# Autodesk Inventor assembly: 1103 Lift - BottomTier
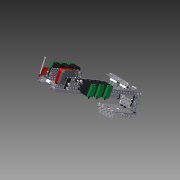
[picture p0: Inventor's stored thumbnail of the model, 180x180]
Saved by Autodesk Inventor 2012 (Build 160160000, 160)
## iProperties
Created: 2011-08-16
Part Number: 1103 Lift - BottomTier
Document SubType Name: Assembly
Designer: Dakota.Bayer
Author: Dakota.Bayer
## Documents named in this file (37)
- C:\Users\Wade\Documents\1103 Robot - CAD Assembly\1103 Lift - Bottom Tier.iam
- C:\Users\Wade\Documents\1103 Robot - CAD Assembly\Outside.ipt
- C:\Users\Wade\Documents\1103 Robot - CAD Assembly\Flat Bearing Block.ipt
- C:\Users\Wade\Documents\1103 Robot - CAD Assembly\2 x 12.ipt
- C:\Users\Wade\Documents\1103 Robot - CAD Assembly\1103 lift base.ipt
- C:\Users\Wade\Documents\24C VEX CAD Files\Washers & Spacers\Spacer (Nylon), 0.125''.ipt
- C:\Users\Wade\Documents\24C VEX CAD Files\Motors & Sensors\Optical Shaft (Quadrature) Encoder.iam
- C:\Users\Wade\Documents\24C VEX CAD Files\Standoffs & Couplers\Standoff 2.40''.ipt
- C:\Users\Wade\Documents\24C VEX CAD Files\Screws & Nuts\Screw 6-32 x 0.250''-Silver.ipt
- C:\Users\Wade\Documents\1103 Robot - CAD Assembly\Bearing Assembly (end hole).iam
- C:\Users\Wade\Documents\1103 Robot - CAD Assembly\Bearing Assembly (both end holes).iam
- C:\Users\Wade\Documents\24C VEX CAD Files\Screws & Nuts\Screw 8-32 x 0.875''-Silver.ipt
- C:\Users\Wade\Documents\24C VEX CAD Files\Screws & Nuts\Nut 8-32 Nylock.ipt
- C:\Users\Wade\Documents\24C VEX CAD Files\Screws & Nuts\Screw 8-32 x 0.500''-Silver.ipt
- C:\Users\Wade\Documents\1103 Robot - CAD Assembly\BEAM-0500.ipt
- C:\Users\Wade\Documents\24C VEX CAD Files\Motors & Sensors\2-Wire Motor 269-Without Wire.iam
- C:\Users\Wade\Documents\1103 Robot - CAD Assembly\VEX-HINGE-2 RevA_1.ipt
- C:\Users\Wade\Documents\1103 Robot - CAD Assembly\1103 sprocket4.ipt
- C:\Users\Wade\Documents\1103 Robot - CAD Assembly\1103 sprocket3.ipt
- C:\Users\Wade\Documents\1103 Robot - CAD Assembly\5 x 2.ipt
- C:\Users\Wade\Documents\1103 Robot - CAD Assembly\1103 sprocket1.ipt
- C:\Users\Wade\Documents\1103 Robot - CAD Assembly\1103 sprocket2.ipt
- C:\Users\Wade\Documents\24C VEX CAD Files\Screws & Nuts\Screw 8-32 x 0.375''-Silver.ipt
- C:\Users\Wade\Documents\1103 Robot - CAD Assembly\.375'' Screw & Nylock Nut.iam
- C:\Users\Wade\Documents\24C VEX CAD Files\Screws & Nuts\Screw 8-32 x 0.250''-Silver.ipt
- C:\Users\Wade\Documents\24C VEX CAD Files\Screws & Nuts\Nut 8-32 Keps.ipt
- C:\Users\Wade\Documents\24C VEX CAD Files\Metal Chassis Rails\Aluminum Chassis Rail 2x1x5.ipt
- C:\Users\Wade\Documents\24C VEX CAD Files\Motors & Sensors\Limit Switch (Sensor).iam
- C:\Users\Wade\Documents\24C VEX CAD Files\Washers & Spacers\Spacer (Thin), 4.6mm.ipt
- C:\Users\Wade\Documents\24C VEX CAD Files\Washers & Spacers\Spacer (Nylon), 0.250''.ipt
- C:\Users\Wade\Documents\24C VEX CAD Files\Standoffs & Couplers\Standoff 0.75''.ipt
- C:\Users\Wade\Documents\24C VEX CAD Files\Screws & Nuts\Screw 6-32 x 0.500''-Silver.ipt
- C:\Users\Wade\Documents\1103 Robot - CAD Assembly\VEX-HINGE 4x RevA.ipt
- C:\Users\Wade\Documents\24C VEX CAD Files\Washers & Spacers\Spacer (Nylon), 0.500'' (mod).ipt
- C:\Users\Wade\Documents\24C VEX CAD Files\Washers & Spacers\Spacer (Nylon), 0.250'' (mod).ipt
- C:\Users\Wade\Documents\24C VEX CAD Files\Other Parts\Bearing Flat (2-hole).ipt
- C:\Users\Wade\Documents\1103 Robot - CAD Assembly\.5'' Screw & Nylock Nut.iam
## Components (141 placed, 36 different names)
1. Outside:3 — Flush:21, Flush:23, Mate:622, Mate:685
2. Outside:4 — Mate:54, Flush:23, Flush:35, Mate:686
3. 1103 lift base:1 — Mate:54, Flush:21, Mate:112, Mate:113, Flush:29, Flush:30, Flush:31, Flush:32, Mate:622, Flush:35, Tangent:152, Mate:633, Tangent:153, Flush:36, Mate:638, Mate:640, Mate:655, Mate:660, Mate:689, Mate:690, Mate:693, Flush:38, Mate:694, Flush:39, Flush:40, Tangent:177, Mate:784, Tangent:219, Tangent:220, Mate:790, Mate:791, Mate:792, Mate:793, Mate:798, Mate:799, Mate:800, Mate:801, Tangent:222, Tangent:223, Tangent:224, Mate:804, Mate:806, Mate:810, Mate:820, Angle:1, Angle:2, Mate:835, Mate:839
4. Screw 8-32 x 0.375''-Silver:1 — Mate:683
5. Screw 8-32 x 0.375''-Silver:2 — Mate:684
6. Screw 8-32 x 0.375''-Silver:3 — Mate:688
7. Screw 8-32 x 0.375''-Silver:4 — Mate:687
8. 2 x 12:1 — Mate:112, Flush:29, Flush:32, Mate:114, Tangent:154, Tangent:155, Tangent:156, Mate:641, Tangent:157, Tangent:158, Tangent:159, Tangent:160, Tangent:161, Mate:644, Mate:661, Mate:674, Mate:675, Mate:676, Mate:816, Mate:817
9. 2 x 12:2 — Mate:113, Flush:30, Flush:31, Mate:119, Mate:625, Mate:645, Mate:648, Tangent:162, Tangent:163, Tangent:164, Tangent:165, Tangent:166, Mate:649, Tangent:167, Mate:654, Mate:667, Mate:668, Mate:669, Mate:818
10. Flat Bearing Block:5 — Mate:114, Mate:664, Flush:37, Mate:741
11. Screw 8-32 x 0.500''-Silver:1 — Mate:661, Mate:662
12. Screw 8-32 x 0.500''-Silver:2 — Mate:660, Mate:663
13. Screw 8-32 x 0.500''-Silver:3 — Mate:654, Mate:657
14. Screw 8-32 x 0.500''-Silver:4 — Mate:655, Mate:656
15. Flat Bearing Block:6 — Mate:119, Mate:658, Mate:659
16. Screw 8-32 x 0.875''-Silver:1 — Mate:691
17. Screw 6-32 x 0.500''-Silver:1
18. Screw 6-32 x 0.500''-Silver:2
19. Screw 6-32 x 0.500''-Silver:3
20. Screw 6-32 x 0.500''-Silver:4
21. Bearing Assembly (end hole):2 [sub-assembly] — Tangent:157, Tangent:158, Mate:816, Mate:817
22. Screw 6-32 x 0.500''-Silver:5
23. Screw 6-32 x 0.500''-Silver:6
24. Screw 6-32 x 0.500''-Silver:7
25. Screw 6-32 x 0.500''-Silver:8
26. Screw 6-32 x 0.500''-Silver:9
27. Screw 6-32 x 0.500''-Silver:10
28. Screw 6-32 x 0.500''-Silver:11
29. Screw 6-32 x 0.500''-Silver:12
30. Spacer (Nylon), 0.125'':1 — Mate:625, Mate:632
31. Optical Shaft (Quadrature) Encoder:1 [sub-assembly] — Mate:632
32. Standoff 2.40'':1 — Tangent:152, Mate:633, Tangent:153, Mate:637, Mate:639
33. Spacer (Nylon), 0.500'' (mod):1 — Flush:36
34. Screw 6-32 x 0.250''-Silver:1 — Mate:639, Mate:640
35. Screw 6-32 x 0.250''-Silver:2 — Mate:637, Mate:638
36. Bearing Assembly (end hole):1 [sub-assembly] — Tangent:154, Tangent:155, Tangent:156, Mate:641
37. Bearing Assembly (end hole):3 [sub-assembly] — Tangent:159, Tangent:160, Tangent:161, Mate:644, Mate:647
38. Bearing Assembly (end hole):5 [sub-assembly] — Mate:648, Tangent:162, Tangent:163, Tangent:164
39. Bearing Assembly (end hole):6 [sub-assembly] — Tangent:165, Tangent:166, Mate:649, Tangent:167
40. Bearing Assembly (both end holes):1 [sub-assembly] — Mate:645, Mate:647, Mate:692, Mate:818
41. Nut 8-32 Nylock:3 — Mate:657, Mate:658
42. Nut 8-32 Nylock:4 — Mate:656, Mate:659
43. BEAM-0500:1 — Mate:662, Flush:37, Mate:740, Mate:742
44. BEAM-0500:2 — Mate:663, Mate:664, Mate:743
45. 2-Wire Motor 269-Without Wire:1 [sub-assembly] — Mate:667
46. 2-Wire Motor 269-Without Wire:2 [sub-assembly] — Mate:669
47. 2-Wire Motor 269-Without Wire:3 [sub-assembly] — Mate:668
48. 2-Wire Motor 269-Without Wire:4 [sub-assembly] — Mate:675
49. 2-Wire Motor 269-Without Wire:5 [sub-assembly] — Mate:676
50. 2-Wire Motor 269-Without Wire:6 [sub-assembly] — Mate:674
51. VEX-HINGE 4x RevA:1 — Mate:802, Mate:803, Mate:822, Angle:2
52. VEX-HINGE-2 RevA_1:1 — Mate:747, Flush:54, Flush:55, Mate:750, Tangent:207, Tangent:209, Tangent:210, Mate:751, Mate:802, Mate:803
53. 1103 sprocket4:1 — Mate:694, Flush:39, Tangent:171, Tangent:172, Tangent:173, Mate:697, Mate:701, Mate:703, Flush:41, Mate:704, Flush:42, Tangent:178, Mate:705, Tangent:179, Tangent:180, Tangent:181
54. 1103 sprocket3:1 — Mate:693, Flush:38, Flush:40, Tangent:168, Tangent:169, Mate:696, Tangent:170, Tangent:174, Tangent:175, Mate:698, Tangent:176, Mate:699, Mate:707, Tangent:182, Tangent:183, Mate:819
55. 5 x 2:1 — Mate:747, Flush:54, Flush:55, Tangent:205, Tangent:206, Tangent:208, Tangent:211, Tangent:212, Tangent:213, Tangent:214, Tangent:215, Tangent:216, Tangent:217, Tangent:218, Mate:776, Mate:777, Mate:778, Mate:779, Mate:780, Mate:782, Mate:783, Mate:785, Mate:821, Mate:822, Angle:1
56. 1103 sprocket1:1 — Mate:709, Flush:43, Flush:44, Mate:722, Tangent:194, Tangent:195, Mate:723, Mate:727, Tangent:198, Tangent:199, Mate:730, Tangent:201, Mate:731, Mate:738, Mate:739
57. 1103 sprocket2:1 — Mate:710, Flush:45, Flush:46, Flush:48, Flush:49, Mate:728, Mate:729, Tangent:196, Tangent:197, Tangent:200, Tangent:202, Mate:736, Mate:737, Mate:831
58. 5 x 2:2 — Flush:41, Mate:704, Flush:42, Tangent:184, Tangent:185, Mate:709, Flush:43, Flush:44, Mate:710, Flush:45, Flush:46, Mate:706, Mate:708, Mate:715, Mate:717, Mate:719, Mate:721, Mate:819, Mate:827, Mate:828, Mate:829, Mate:830
59. Nut 8-32 Nylock:5 — Mate:684, Mate:686
60. Nut 8-32 Nylock:6 — Mate:683, Mate:685
61. Nut 8-32 Nylock:7 — Mate:688, Mate:689
62. Nut 8-32 Nylock:8 — Mate:687, Mate:690
63. Nut 8-32 Nylock:9 — Mate:691, Mate:692
64. Bearing Assembly (both end holes):2 [sub-assembly] — Tangent:168, Tangent:169, Mate:696, Tangent:170
65. Bearing Assembly (both end holes):3 [sub-assembly] — Tangent:171, Tangent:172, Tangent:173, Mate:697
66. .375'' Screw & Nylock Nut:1 [sub-assembly] — Tangent:176, Tangent:177, Mate:699, Mate:700
67. .375'' Screw & Nylock Nut:2 [sub-assembly] — Mate:702, Mate:703
68. .375'' Screw & Nylock Nut:3 [sub-assembly] — Mate:700, Mate:701
69. .375'' Screw & Nylock Nut:4 [sub-assembly] — Tangent:174, Tangent:175, Mate:698, Mate:702
70. .375'' Screw & Nylock Nut:5 [sub-assembly] — Tangent:178, Mate:705, Tangent:179
71. .375'' Screw & Nylock Nut:6 [sub-assembly] — Mate:706, Tangent:180, Tangent:181
72. .375'' Screw & Nylock Nut:7 [sub-assembly] — Mate:707, Tangent:184, Tangent:185
73. .375'' Screw & Nylock Nut:8 [sub-assembly] — Mate:708, Tangent:182, Tangent:183
74. Screw 8-32 x 0.375''-Silver:5
75. Screw 8-32 x 0.375''-Silver:6 — Mate:831
76. Screw 8-32 x 0.375''-Silver:8
77. Screw 8-32 x 0.375''-Silver:7
78. Nut 8-32 Keps:1 — Mate:715
79. Nut 8-32 Keps:2 — Mate:721
80. Nut 8-32 Keps:3 — Mate:719
81. Nut 8-32 Keps:4 — Mate:717
82. Aluminum Chassis Rail 2x1x5:1 — Flush:48, Mate:722, Flush:49, Flush:50
83. .375'' Screw & Nylock Nut:9 [sub-assembly] — Tangent:194, Tangent:195, Mate:723
84. .375'' Screw & Nylock Nut:10 [sub-assembly] — Mate:725, Mate:727, Tangent:198
85. .375'' Screw & Nylock Nut:11 [sub-assembly] — Mate:724, Mate:729, Tangent:196
86. .375'' Screw & Nylock Nut:12 [sub-assembly] — Mate:726, Mate:728, Tangent:197
87. Standoff 2.40'':2 — Tangent:199, Mate:730, Tangent:200, Mate:732, Mate:735
88. Standoff 2.40'':3 — Tangent:201, Tangent:202, Mate:731, Mate:733, Mate:734
89. Screw 8-32 x 0.250''-Silver:5 — Mate:733, Mate:738
90. Screw 8-32 x 0.250''-Silver:6 — Mate:732, Mate:739
91. Screw 8-32 x 0.250''-Silver:7 — Mate:734, Mate:736
92. Screw 8-32 x 0.250''-Silver:8 — Mate:735, Mate:737
93. Limit Switch (Sensor):1 [sub-assembly] — Mate:740, Mate:741, Mate:744, Mate:745
94. Screw 8-32 x 0.500''-Silver:5 — Mate:743, Mate:745
95. Screw 8-32 x 0.500''-Silver:6 — Mate:742, Mate:744
96. Spacer (Thin), 4.6mm:1 — Flush:59, Mate:752, Mate:766, Mate:771
97. Spacer (Nylon), 0.250'':1 — Tangent:211, Tangent:212, Flush:59, Mate:754, Mate:764, Mate:821
98. Spacer (Thin), 4.6mm:2 — Tangent:205, Tangent:206, Flush:58, Mate:753, Mate:772, Mate:781
99. Spacer (Nylon), 0.250'' (mod):1 — Tangent:213, Tangent:214, Flush:58, Mate:755, Mate:765
100. Spacer (Thin), 4.6mm:3 — Tangent:207, Tangent:208, Mate:750, Flush:57, Mate:756, Mate:763, Mate:773
101. Spacer (Nylon), 0.250'':3 — Tangent:217, Tangent:218, Flush:56, Mate:759, Mate:760, Mate:767
102. Spacer (Thin), 4.6mm:4 — Tangent:209, Tangent:210, Mate:751, Flush:56, Mate:757, Mate:762, Mate:770
103. Spacer (Nylon), 0.250'' (mod):2 — Tangent:215, Tangent:216, Flush:57, Mate:758, Mate:761
104. Standoff 0.75'':1 — Mate:752, Mate:766, Mate:788
105. Standoff 0.75'':2 — Mate:753, Mate:781, Mate:784, Mate:789
106. Standoff 0.75'':3 — Mate:754, Mate:764, Mate:769, Tangent:219, Tangent:220, Mate:786, Mate:820
107. Standoff 0.75'':4 — Mate:755, Mate:765, Mate:787
108. Standoff 0.75'':5 — Mate:756, Mate:763, Mate:796
109. Standoff 0.75'':6 — Mate:757, Mate:762, Mate:797
110. Standoff 0.75'':7 — Mate:758, Mate:761, Mate:774, Mate:794
111. Standoff 0.75'':8 — Mate:759, Mate:760, Mate:795
112. Screw 8-32 x 0.500''-Silver:7 — Mate:767, Mate:777
113. Screw 8-32 x 0.500''-Silver:8 — Mate:783
114. Screw 8-32 x 0.500''-Silver:9 — Mate:769, Mate:782
115. Screw 8-32 x 0.500''-Silver:10 — Mate:770, Mate:778
116. Screw 8-32 x 0.500''-Silver:11 — Mate:773, Mate:779
117. Screw 8-32 x 0.500''-Silver:12 — Mate:772, Mate:780
118. Screw 8-32 x 0.500''-Silver:13 — Mate:774, Mate:776
119. Screw 8-32 x 0.500''-Silver:14 — Mate:771, Mate:785
120. Screw 8-32 x 0.250''-Silver:9 — Mate:786, Mate:790
121. Screw 8-32 x 0.250''-Silver:10 — Mate:787, Mate:791
122. Screw 8-32 x 0.250''-Silver:11 — Mate:788, Mate:793
123. Screw 8-32 x 0.250''-Silver:12 — Mate:789, Mate:792
124. Screw 8-32 x 0.250''-Silver:13 — Mate:794, Mate:799
125. Screw 8-32 x 0.250''-Silver:14 — Mate:795, Mate:800
126. Screw 8-32 x 0.250''-Silver:15 — Mate:796, Mate:798
127. Screw 8-32 x 0.250''-Silver:16 — Mate:797, Mate:801
128. Bearing Flat (2-hole):1 — Tangent:222, Tangent:223, Tangent:224, Mate:804, Mate:805, Mate:807, Mate:808, Mate:811, Mate:812, Mate:813
129. Bearing Flat (2-hole):2 — Mate:805, Mate:806, Mate:807, Mate:809, Mate:814, Mate:815
130. .5'' Screw & Nylock Nut:1 [sub-assembly] — Mate:808, Mate:811
131. .5'' Screw & Nylock Nut:2 [sub-assembly] — Mate:809, Mate:810
132. Spacer (Thin), 4.6mm:5 — Mate:812, Mate:813, Mate:836, Mate:837
133. Spacer (Thin), 4.6mm:6 — Mate:814, Mate:815, Mate:832, Mate:834
134. Spacer (Thin), 4.6mm:7 — Mate:827
135. Spacer (Thin), 4.6mm:8 — Mate:828
136. Spacer (Thin), 4.6mm:9 — Mate:829
137. Spacer (Thin), 4.6mm:10 — Mate:830
138. Nut 8-32 Nylock:10 — Mate:833, Mate:835
139. Screw 8-32 x 0.875''-Silver:2 — Mate:832, Mate:833, Mate:834
140. Nut 8-32 Nylock:11 — Mate:838, Mate:839
141. Screw 8-32 x 0.875''-Silver:3 — Mate:836, Mate:837, Mate:838
## Relationships (363: Mate 220, Tangent 114, Flush 27, Angle 2)
- Mate:54: Outside:4 ↔ 1103 lift base:1
- Flush:21: Outside:3 ↔ 1103 lift base:1
- [Tangent] (0.2286 mm): 1103 lift base:1 ↔ Screw 8-32 x 0.375''-Silver:1
- [Tangent] (0.2286 mm): 1103 lift base:1 ↔ Screw 8-32 x 0.375''-Silver:2
- [Mate]: Outside:4 ↔ Screw 8-32 x 0.375''-Silver:3
- [Mate]: Outside:3 ↔ Screw 8-32 x 0.375''-Silver:4
- [Tangent] (0.2286 mm): 1103 lift base:1 ↔ Screw 8-32 x 0.375''-Silver:4
- [Tangent] (0.2286 mm): 1103 lift base:1 ↔ Screw 8-32 x 0.375''-Silver:3
- [Tangent] (0.2286 mm): 1103 lift base:1 ↔ Screw 8-32 x 0.375''-Silver:1
- [Tangent] (0.2286 mm): Outside:3 ↔ Screw 8-32 x 0.375''-Silver:1
- [Tangent] (0.2286 mm): 1103 lift base:1 ↔ Screw 8-32 x 0.375''-Silver:2
- [Tangent] (0.2286 mm): Outside:4 ↔ Screw 8-32 x 0.375''-Silver:2
- [Tangent] (0.2286 mm): Outside:4 ↔ Screw 8-32 x 0.375''-Silver:3
- [Tangent] (0.2286 mm): Outside:3 ↔ Screw 8-32 x 0.375''-Silver:4
- Flush:23: Outside:3 ↔ Outside:4
- Mate:112: 1103 lift base:1 ↔ 2 x 12:1
- Mate:113: 1103 lift base:1 ↔ 2 x 12:2
- Flush:29: 1103 lift base:1 ↔ 2 x 12:1
- Flush:30: 1103 lift base:1 ↔ 2 x 12:2
- Flush:31: 1103 lift base:1 ↔ 2 x 12:2
- Flush:32: 1103 lift base:1 ↔ 2 x 12:1
- Mate:114: 2 x 12:1 ↔ Flat Bearing Block:5
- [Tangent] (0.2286 mm): 2 x 12:1 ↔ Screw 8-32 x 0.500''-Silver:2
- [Tangent] (0.2286 mm): 2 x 12:1 ↔ Screw 8-32 x 0.500''-Silver:2
- [Tangent] (0.2286 mm): 2 x 12:1 ↔ Screw 8-32 x 0.500''-Silver:1
- [Tangent] (0.2286 mm): 2 x 12:1 ↔ Screw 8-32 x 0.500''-Silver:1
- [Mate]: Flat Bearing Block:5 ↔ Screw 8-32 x 0.500''-Silver:1
- [Mate]: Flat Bearing Block:5 ↔ Screw 8-32 x 0.500''-Silver:2
- Mate:119: 2 x 12:2 ↔ Flat Bearing Block:6
- [Tangent] (0.2286 mm): 1103 lift base:1 ↔ Screw 8-32 x 0.500''-Silver:4
- [Tangent] (0.2286 mm): 2 x 12:2 ↔ Screw 8-32 x 0.500''-Silver:4
- [Tangent] (0.2286 mm): 2 x 12:2 ↔ Screw 8-32 x 0.500''-Silver:3
- [Tangent] (0.2286 mm): 2 x 12:2 ↔ Screw 8-32 x 0.500''-Silver:3
- [Mate]: Screw 8-32 x 0.500''-Silver:3 ↔ Flat Bearing Block:6
- [Mate]: Screw 8-32 x 0.500''-Silver:4 ↔ Flat Bearing Block:6
- [Mate]: 2 x 12:2 ↔ Screw 6-32 x 0.500''-Silver:1
- [Mate]: 1103 lift base:1 ↔ Screw 6-32 x 0.500''-Silver:2
- [Mate]: 2 x 12:1 ↔ Screw 6-32 x 0.500''-Silver:4
- [Mate]: 2 x 12:1 ↔ Screw 6-32 x 0.500''-Silver:3
- [Tangent] (0.4572 mm): 2 x 12:1 ↔ Screw 6-32 x 0.500''-Silver:3
- [Tangent] (0.4572 mm): 2 x 12:1 ↔ Screw 6-32 x 0.500''-Silver:3
- [Tangent] (0.4572 mm): 2 x 12:1 ↔ Screw 6-32 x 0.500''-Silver:4
- [Tangent] (0.4572 mm): 2 x 12:1 ↔ Screw 6-32 x 0.500''-Silver:4
- [Tangent] (0.4572 mm): 2 x 12:2 ↔ Screw 6-32 x 0.500''-Silver:1
- [Tangent] (0.4572 mm): 2 x 12:2 ↔ Screw 6-32 x 0.500''-Silver:1
- [Tangent] (0.4572 mm): 1103 lift base:1 ↔ Screw 6-32 x 0.500''-Silver:2
- [Tangent] (0.4572 mm): 1103 lift base:1 ↔ Screw 6-32 x 0.500''-Silver:2
- [Mate]: 2 x 12:2 ↔ Screw 6-32 x 0.500''-Silver:5
- [Mate]: 1103 lift base:1 ↔ Screw 6-32 x 0.500''-Silver:6
- [Mate]: 2 x 12:2 ↔ Screw 6-32 x 0.500''-Silver:8
- [Mate]: 1103 lift base:1 ↔ Screw 6-32 x 0.500''-Silver:7
- [Tangent] (0.4572 mm): 2 x 12:2 ↔ Screw 6-32 x 0.500''-Silver:5
- [Tangent] (0.4572 mm): 2 x 12:2 ↔ Screw 6-32 x 0.500''-Silver:5
- [Tangent] (0.4572 mm): 2 x 12:2 ↔ Screw 6-32 x 0.500''-Silver:6
- [Tangent] (0.4572 mm): 2 x 12:2 ↔ Screw 6-32 x 0.500''-Silver:6
- [Tangent] (0.4572 mm): 2 x 12:2 ↔ Screw 6-32 x 0.500''-Silver:7
- [Tangent] (0.4572 mm): 2 x 12:2 ↔ Screw 6-32 x 0.500''-Silver:7
- [Tangent] (0.4572 mm): 2 x 12:2 ↔ Screw 6-32 x 0.500''-Silver:8
- [Tangent] (0.4572 mm): 2 x 12:2 ↔ Screw 6-32 x 0.500''-Silver:8
- [Mate]: 2 x 12:1 ↔ Screw 6-32 x 0.500''-Silver:12
- [Mate]: 1103 lift base:1 ↔ Screw 6-32 x 0.500''-Silver:11
- [Mate]: 2 x 12:1 ↔ Screw 6-32 x 0.500''-Silver:10
- [Mate]: 1103 lift base:1 ↔ Screw 6-32 x 0.500''-Silver:9
- [Tangent] (0.4572 mm): 2 x 12:1 ↔ Screw 6-32 x 0.500''-Silver:10
- [Tangent] (0.4572 mm): 2 x 12:1 ↔ Screw 6-32 x 0.500''-Silver:10
- [Tangent] (0.4572 mm): 2 x 12:1 ↔ Screw 6-32 x 0.500''-Silver:9
- [Tangent] (0.4572 mm): 2 x 12:1 ↔ Screw 6-32 x 0.500''-Silver:9
- [Tangent] (0.4572 mm): 2 x 12:1 ↔ Screw 6-32 x 0.500''-Silver:12
- [Tangent] (0.4572 mm): 2 x 12:1 ↔ Screw 6-32 x 0.500''-Silver:12
- [Tangent] (0.4572 mm): 2 x 12:1 ↔ Screw 6-32 x 0.500''-Silver:11
- [Tangent] (0.4572 mm): 2 x 12:1 ↔ Screw 6-32 x 0.500''-Silver:11
- Mate:622: Outside:3 ↔ 1103 lift base:1
- [Mate]: Screw 8-32 x 0.875''-Silver:1 ↔ Spacer (Nylon), 0.125'':1
- Mate:625: 2 x 12:2 ↔ Spacer (Nylon), 0.125'':1
- Flush:35: Outside:4 ↔ 1103 lift base:1
- [Tangent] (0.1905 mm): 2 x 12:2 ↔ Screw 8-32 x 0.875''-Silver:1
- Mate:632: Spacer (Nylon), 0.125'':1 ↔ Optical Shaft (Quadrature) Encoder:1
- [Tangent] (0.1905 mm): Screw 8-32 x 0.875''-Silver:1 ↔ Optical Shaft (Quadrature) Encoder:1
- Tangent:152 (0.2311 mm): 1103 lift base:1 ↔ Standoff 2.40'':1
- Mate:633: 1103 lift base:1 ↔ Standoff 2.40'':1
- Tangent:153 (0.2311 mm): 1103 lift base:1 ↔ Standoff 2.40'':1
- [Mate]: 1103 lift base:1 ↔ Screw 8-32 x 0.375''-Silver:2
- [Mate]: 1103 lift base:1 ↔ Screw 8-32 x 0.375''-Silver:1
- Flush:36 (23.876 mm): 1103 lift base:1 ↔ Spacer (Nylon), 0.500'' (mod):1
- Mate:637: Standoff 2.40'':1 ↔ Screw 6-32 x 0.250''-Silver:2
- Mate:638: 1103 lift base:1 ↔ Screw 6-32 x 0.250''-Silver:2
- Mate:639: Standoff 2.40'':1 ↔ Screw 6-32 x 0.250''-Silver:1
- Mate:640: 1103 lift base:1 ↔ Screw 6-32 x 0.250''-Silver:1
- Tangent:154 (0.2311 mm): 2 x 12:1 ↔ Bearing Assembly (end hole):1
- Tangent:155 (0.2311 mm): 2 x 12:1 ↔ Bearing Assembly (end hole):1
- Tangent:156 (0.2311 mm): 2 x 12:1 ↔ Bearing Assembly (end hole):1
- Mate:641: 2 x 12:1 ↔ Bearing Assembly (end hole):1
- Tangent:157 (0.1905 mm): 2 x 12:1 ↔ Bearing Assembly (end hole):2
- Tangent:158 (0.1905 mm): 2 x 12:1 ↔ Bearing Assembly (end hole):2
- Tangent:159 (0.1905 mm): 2 x 12:1 ↔ Bearing Assembly (end hole):3
- Tangent:160 (0.1905 mm): 2 x 12:1 ↔ Bearing Assembly (end hole):3
- Tangent:161 (0.1905 mm): 2 x 12:1 ↔ Bearing Assembly (end hole):3
- Mate:644: 2 x 12:1 ↔ Bearing Assembly (end hole):3
- Mate:645: 2 x 12:2 ↔ Bearing Assembly (both end holes):1
- Mate:647: Bearing Assembly (end hole):3 ↔ Bearing Assembly (both end holes):1
- Mate:648: 2 x 12:2 ↔ Bearing Assembly (end hole):5
- Tangent:162 (0.2311 mm): 2 x 12:2 ↔ Bearing Assembly (end hole):5
- Tangent:163 (0.2311 mm): 2 x 12:2 ↔ Bearing Assembly (end hole):5
- Tangent:164 (0.2311 mm): 2 x 12:2 ↔ Bearing Assembly (end hole):5
- Tangent:165 (0.2311 mm): 2 x 12:2 ↔ Bearing Assembly (end hole):6
- Tangent:166 (0.2311 mm): 2 x 12:2 ↔ Bearing Assembly (end hole):6
- Mate:649: 2 x 12:2 ↔ Bearing Assembly (end hole):6
- Tangent:167 (0.2311 mm): 2 x 12:2 ↔ Bearing Assembly (end hole):6
- Mate:654: 2 x 12:2 ↔ Screw 8-32 x 0.500''-Silver:3
- Mate:655: 1103 lift base:1 ↔ Screw 8-32 x 0.500''-Silver:4
- Mate:656: Screw 8-32 x 0.500''-Silver:4 ↔ Nut 8-32 Nylock:4
- Mate:657: Screw 8-32 x 0.500''-Silver:3 ↔ Nut 8-32 Nylock:3
- Mate:658: Flat Bearing Block:6 ↔ Nut 8-32 Nylock:3
- Mate:659: Flat Bearing Block:6 ↔ Nut 8-32 Nylock:4
- Mate:660: 1103 lift base:1 ↔ Screw 8-32 x 0.500''-Silver:2
- Mate:661: 2 x 12:1 ↔ Screw 8-32 x 0.500''-Silver:1
- Mate:662: Screw 8-32 x 0.500''-Silver:1 ↔ BEAM-0500:1
- Mate:663: Screw 8-32 x 0.500''-Silver:2 ↔ BEAM-0500:2
- Mate:664: Flat Bearing Block:5 ↔ BEAM-0500:2
- Flush:37 (-12.7 mm): Flat Bearing Block:5 ↔ BEAM-0500:1
- [Mate]: Screw 6-32 x 0.500''-Silver:2 ↔ 2-Wire Motor 269-Without Wire:1
- [Mate]: Screw 6-32 x 0.500''-Silver:1 ↔ 2-Wire Motor 269-Without Wire:1
- Mate:667: 2 x 12:2 ↔ 2-Wire Motor 269-Without Wire:1
- Mate:668: 2 x 12:2 ↔ 2-Wire Motor 269-Without Wire:3
- Mate:669: 2 x 12:2 ↔ 2-Wire Motor 269-Without Wire:2
- [Mate]: Screw 6-32 x 0.500''-Silver:7 ↔ 2-Wire Motor 269-Without Wire:2
- [Mate]: Screw 6-32 x 0.500''-Silver:8 ↔ 2-Wire Motor 269-Without Wire:2
- [Mate]: Screw 6-32 x 0.500''-Silver:6 ↔ 2-Wire Motor 269-Without Wire:3
- [Mate]: Screw 6-32 x 0.500''-Silver:5 ↔ 2-Wire Motor 269-Without Wire:3
- Mate:674: 2 x 12:1 ↔ 2-Wire Motor 269-Without Wire:6
- Mate:675: 2 x 12:1 ↔ 2-Wire Motor 269-Without Wire:4
- Mate:676: 2 x 12:1 ↔ 2-Wire Motor 269-Without Wire:5
- [Mate]: Screw 6-32 x 0.500''-Silver:3 ↔ 2-Wire Motor 269-Without Wire:5
- [Mate]: Screw 6-32 x 0.500''-Silver:4 ↔ 2-Wire Motor 269-Without Wire:5
- [Mate]: Screw 6-32 x 0.500''-Silver:9 ↔ 2-Wire Motor 269-Without Wire:6
- [Mate]: Screw 6-32 x 0.500''-Silver:10 ↔ 2-Wire Motor 269-Without Wire:6
- [Mate]: Screw 6-32 x 0.500''-Silver:12 ↔ 2-Wire Motor 269-Without Wire:4
- [Mate]: Screw 6-32 x 0.500''-Silver:11 ↔ 2-Wire Motor 269-Without Wire:4
- Mate:683: Screw 8-32 x 0.375''-Silver:1 ↔ Nut 8-32 Nylock:6
- Mate:684: Screw 8-32 x 0.375''-Silver:2 ↔ Nut 8-32 Nylock:5
- Mate:685: Outside:3 ↔ Nut 8-32 Nylock:6
- Mate:686: Outside:4 ↔ Nut 8-32 Nylock:5
- Mate:687: Screw 8-32 x 0.375''-Silver:4 ↔ Nut 8-32 Nylock:8
- Mate:688: Screw 8-32 x 0.375''-Silver:3 ↔ Nut 8-32 Nylock:7
- Mate:689: 1103 lift base:1 ↔ Nut 8-32 Nylock:7
- Mate:690: 1103 lift base:1 ↔ Nut 8-32 Nylock:8
- Mate:691: Screw 8-32 x 0.875''-Silver:1 ↔ Nut 8-32 Nylock:9
- Mate:692: Bearing Assembly (both end holes):1 ↔ Nut 8-32 Nylock:9
- Mate:693: 1103 lift base:1 ↔ 1103 sprocket3:1
- Flush:38: 1103 lift base:1 ↔ 1103 sprocket3:1
- Mate:694: 1103 lift base:1 ↔ 1103 sprocket4:1
- Flush:39: 1103 lift base:1 ↔ 1103 sprocket4:1
- Flush:40: 1103 lift base:1 ↔ 1103 sprocket3:1
- Tangent:168 (0.2311 mm): 1103 sprocket3:1 ↔ Bearing Assembly (both end holes):2
- Tangent:169 (0.2311 mm): 1103 sprocket3:1 ↔ Bearing Assembly (both end holes):2
- Mate:696: 1103 sprocket3:1 ↔ Bearing Assembly (both end holes):2
- Tangent:170 (0.2311 mm): 1103 sprocket3:1 ↔ Bearing Assembly (both end holes):2
- Tangent:171 (0.2311 mm): 1103 sprocket4:1 ↔ Bearing Assembly (both end holes):3
- Tangent:172 (0.2311 mm): 1103 sprocket4:1 ↔ Bearing Assembly (both end holes):3
- Tangent:173 (0.2311 mm): 1103 sprocket4:1 ↔ Bearing Assembly (both end holes):3
- Mate:697: 1103 sprocket4:1 ↔ Bearing Assembly (both end holes):3
- Tangent:174 (0.2311 mm): 1103 sprocket3:1 ↔ .375'' Screw & Nylock Nut:4
- Tangent:175 (0.2311 mm): 1103 sprocket3:1 ↔ .375'' Screw & Nylock Nut:4
- Mate:698: 1103 sprocket3:1 ↔ .375'' Screw & Nylock Nut:4
- Tangent:176 (0.2311 mm): 1103 sprocket3:1 ↔ .375'' Screw & Nylock Nut:1
- Tangent:177 (0.2311 mm): 1103 lift base:1 ↔ .375'' Screw & Nylock Nut:1
- Mate:699: 1103 sprocket3:1 ↔ .375'' Screw & Nylock Nut:1
- Mate:700: .375'' Screw & Nylock Nut:1 ↔ .375'' Screw & Nylock Nut:3
- Mate:701: 1103 sprocket4:1 ↔ .375'' Screw & Nylock Nut:3
- Mate:702: .375'' Screw & Nylock Nut:2 ↔ .375'' Screw & Nylock Nut:4
- Mate:703: 1103 sprocket4:1 ↔ .375'' Screw & Nylock Nut:2
- Flush:41: 1103 sprocket4:1 ↔ 5 x 2:2
- Mate:704: 1103 sprocket4:1 ↔ 5 x 2:2
- Flush:42: 1103 sprocket4:1 ↔ 5 x 2:2
- Tangent:178 (0.2311 mm): 1103 sprocket4:1 ↔ .375'' Screw & Nylock Nut:5
- Mate:705: 1103 sprocket4:1 ↔ .375'' Screw & Nylock Nut:5
- Tangent:179 (0.2311 mm): 1103 sprocket4:1 ↔ .375'' Screw & Nylock Nut:5
- Mate:706: 5 x 2:2 ↔ .375'' Screw & Nylock Nut:6
- Tangent:180 (0.2311 mm): 1103 sprocket4:1 ↔ .375'' Screw & Nylock Nut:6
- Tangent:181 (0.2311 mm): 1103 sprocket4:1 ↔ .375'' Screw & Nylock Nut:6
- Mate:707: 1103 sprocket3:1 ↔ .375'' Screw & Nylock Nut:7
- Mate:708: 5 x 2:2 ↔ .375'' Screw & Nylock Nut:8
- Tangent:182 (0.2311 mm): 1103 sprocket3:1 ↔ .375'' Screw & Nylock Nut:8
- Tangent:183 (0.2311 mm): 1103 sprocket3:1 ↔ .375'' Screw & Nylock Nut:8
- Tangent:184 (0.2311 mm): 5 x 2:2 ↔ .375'' Screw & Nylock Nut:7
- Tangent:185: 5 x 2:2 ↔ .375'' Screw & Nylock Nut:7
- Mate:709 (4.5974 mm): 1103 sprocket1:1 ↔ 5 x 2:2
- Flush:43: 1103 sprocket1:1 ↔ 5 x 2:2
- Flush:44: 1103 sprocket1:1 ↔ 5 x 2:2
- Mate:710 (4.5974 mm): 1103 sprocket2:1 ↔ 5 x 2:2
- Flush:45: 1103 sprocket2:1 ↔ 5 x 2:2
- Flush:46: 1103 sprocket2:1 ↔ 5 x 2:2
- [Tangent] (0.2311 mm): 1103 sprocket2:1 ↔ Screw 8-32 x 0.375''-Silver:5
- [Tangent] (0.2311 mm): 5 x 2:2 ↔ Screw 8-32 x 0.375''-Silver:5
- [Mate]: 1103 sprocket2:1 ↔ Screw 8-32 x 0.375''-Silver:5
- [Tangent] (0.2311 mm): 1103 sprocket2:1 ↔ Screw 8-32 x 0.375''-Silver:6
- [Tangent] (0.2311 mm): 1103 sprocket2:1 ↔ Screw 8-32 x 0.375''-Silver:6
- [Tangent] (0.2311 mm): 1103 sprocket1:1 ↔ Screw 8-32 x 0.375''-Silver:8
- [Tangent] (0.2311 mm): 1103 sprocket1:1 ↔ Screw 8-32 x 0.375''-Silver:8
- [Mate]: 1103 sprocket1:1 ↔ Screw 8-32 x 0.375''-Silver:8
- [Tangent] (0.2311 mm): 1103 sprocket1:1 ↔ Screw 8-32 x 0.375''-Silver:7
- [Tangent] (0.2311 mm): 1103 sprocket1:1 ↔ Screw 8-32 x 0.375''-Silver:7
- [Mate]: 1103 sprocket1:1 ↔ Screw 8-32 x 0.375''-Silver:7
- [Mate]: Screw 8-32 x 0.375''-Silver:5 ↔ Nut 8-32 Keps:1
- Mate:715: 5 x 2:2 ↔ Nut 8-32 Keps:1
- [Mate]: Screw 8-32 x 0.375''-Silver:6 ↔ Nut 8-32 Keps:4
- Mate:717: 5 x 2:2 ↔ Nut 8-32 Keps:4
- [Mate]: Screw 8-32 x 0.375''-Silver:7 ↔ Nut 8-32 Keps:3
- Mate:719: 5 x 2:2 ↔ Nut 8-32 Keps:3
- [Mate]: Screw 8-32 x 0.375''-Silver:8 ↔ Nut 8-32 Keps:2
- Mate:721: 5 x 2:2 ↔ Nut 8-32 Keps:2
- Flush:48: 1103 sprocket2:1 ↔ Aluminum Chassis Rail 2x1x5:1
- Mate:722: 1103 sprocket1:1 ↔ Aluminum Chassis Rail 2x1x5:1
- Flush:49: 1103 sprocket2:1 ↔ Aluminum Chassis Rail 2x1x5:1
- Tangent:194 (0.2311 mm): 1103 sprocket1:1 ↔ .375'' Screw & Nylock Nut:9
- Tangent:195 (0.2311 mm): 1103 sprocket1:1 ↔ .375'' Screw & Nylock Nut:9
- Mate:723: 1103 sprocket1:1 ↔ .375'' Screw & Nylock Nut:9
- Flush:50 (2.3114 mm): Aluminum Chassis Rail 2x1x5:1
- Mate:724: .375'' Screw & Nylock Nut:11
- Mate:725: .375'' Screw & Nylock Nut:10
- Mate:726: .375'' Screw & Nylock Nut:12
- Mate:727: 1103 sprocket1:1 ↔ .375'' Screw & Nylock Nut:10
- Mate:728: 1103 sprocket2:1 ↔ .375'' Screw & Nylock Nut:12
- Mate:729: 1103 sprocket2:1 ↔ .375'' Screw & Nylock Nut:11
- Tangent:196 (0.2311 mm): 1103 sprocket2:1 ↔ .375'' Screw & Nylock Nut:11
- Tangent:197 (0.2311 mm): 1103 sprocket2:1 ↔ .375'' Screw & Nylock Nut:12
- Tangent:198 (0.2311 mm): 1103 sprocket1:1 ↔ .375'' Screw & Nylock Nut:10
- Tangent:199 (0.2311 mm): 1103 sprocket1:1 ↔ Standoff 2.40'':2
- Mate:730: 1103 sprocket1:1 ↔ Standoff 2.40'':2
- Tangent:200 (0.2311 mm): 1103 sprocket2:1 ↔ Standoff 2.40'':2
- Tangent:201 (0.2311 mm): 1103 sprocket1:1 ↔ Standoff 2.40'':3
- Tangent:202 (0.2311 mm): 1103 sprocket2:1 ↔ Standoff 2.40'':3
- Mate:731: 1103 sprocket1:1 ↔ Standoff 2.40'':3
- Mate:732: Standoff 2.40'':2 ↔ Screw 8-32 x 0.250''-Silver:6
- Mate:733: Standoff 2.40'':3 ↔ Screw 8-32 x 0.250''-Silver:5
- Mate:734: Standoff 2.40'':3 ↔ Screw 8-32 x 0.250''-Silver:7
- Mate:735: Standoff 2.40'':2 ↔ Screw 8-32 x 0.250''-Silver:8
- Mate:736: 1103 sprocket2:1 ↔ Screw 8-32 x 0.250''-Silver:7
- Mate:737: 1103 sprocket2:1 ↔ Screw 8-32 x 0.250''-Silver:8
- Mate:738: 1103 sprocket1:1 ↔ Screw 8-32 x 0.250''-Silver:5
- Mate:739: 1103 sprocket1:1 ↔ Screw 8-32 x 0.250''-Silver:6
- Mate:740: BEAM-0500:1 ↔ Limit Switch (Sensor):1
- Mate:741: Flat Bearing Block:5 ↔ Limit Switch (Sensor):1
- Mate:742: BEAM-0500:1 ↔ Screw 8-32 x 0.500''-Silver:6
- Mate:743: BEAM-0500:2 ↔ Screw 8-32 x 0.500''-Silver:5
- Mate:744: Limit Switch (Sensor):1 ↔ Screw 8-32 x 0.500''-Silver:6
- Mate:745: Limit Switch (Sensor):1 ↔ Screw 8-32 x 0.500''-Silver:5
- Mate:747: VEX-HINGE-2 RevA_1:1 ↔ 5 x 2:1
- Flush:54: VEX-HINGE-2 RevA_1:1 ↔ 5 x 2:1
- Flush:55: VEX-HINGE-2 RevA_1:1 ↔ 5 x 2:1
- Tangent:205 (0.2286 mm): 5 x 2:1 ↔ Spacer (Thin), 4.6mm:2
- Tangent:206 (0.2286 mm): 5 x 2:1 ↔ Spacer (Thin), 4.6mm:2
- Tangent:207 (0.2311 mm): VEX-HINGE-2 RevA_1:1 ↔ Spacer (Thin), 4.6mm:3
- Tangent:208 (0.2286 mm): 5 x 2:1 ↔ Spacer (Thin), 4.6mm:3
- Mate:750: VEX-HINGE-2 RevA_1:1 ↔ Spacer (Thin), 4.6mm:3
- Tangent:209 (0.2311 mm): VEX-HINGE-2 RevA_1:1 ↔ Spacer (Thin), 4.6mm:4
- Tangent:210 (0.2311 mm): VEX-HINGE-2 RevA_1:1 ↔ Spacer (Thin), 4.6mm:4
- Mate:751: VEX-HINGE-2 RevA_1:1 ↔ Spacer (Thin), 4.6mm:4
- Tangent:211 (-0.2286 mm): 5 x 2:1 ↔ Spacer (Nylon), 0.250'':1
- Tangent:212 (-0.2286 mm): 5 x 2:1 ↔ Spacer (Nylon), 0.250'':1
- Tangent:213 (-0.2286 mm): 5 x 2:1 ↔ Spacer (Nylon), 0.250'' (mod):1
- Tangent:214 (-0.2286 mm): 5 x 2:1 ↔ Spacer (Nylon), 0.250'' (mod):1
- Tangent:215 (-0.2286 mm): 5 x 2:1 ↔ Spacer (Nylon), 0.250'' (mod):2
- Tangent:216 (-0.2286 mm): 5 x 2:1 ↔ Spacer (Nylon), 0.250'' (mod):2
- Tangent:217 (-0.2286 mm): 5 x 2:1 ↔ Spacer (Nylon), 0.250'':3
- Tangent:218 (-0.2286 mm): 5 x 2:1 ↔ Spacer (Nylon), 0.250'':3
- Flush:56: Spacer (Nylon), 0.250'':3 ↔ Spacer (Thin), 4.6mm:4
- Flush:57: Spacer (Thin), 4.6mm:3 ↔ Spacer (Nylon), 0.250'' (mod):2
- Flush:58: Spacer (Thin), 4.6mm:2 ↔ Spacer (Nylon), 0.250'' (mod):1
- Flush:59: Spacer (Thin), 4.6mm:1 ↔ Spacer (Nylon), 0.250'':1
- Mate:752: Spacer (Thin), 4.6mm:1 ↔ Standoff 0.75'':1
- Mate:753: Spacer (Thin), 4.6mm:2 ↔ Standoff 0.75'':2
- Mate:754: Spacer (Nylon), 0.250'':1 ↔ Standoff 0.75'':3
- Mate:755: Spacer (Nylon), 0.250'' (mod):1 ↔ Standoff 0.75'':4
- Mate:756: Spacer (Thin), 4.6mm:3 ↔ Standoff 0.75'':5
- Mate:757: Spacer (Thin), 4.6mm:4 ↔ Standoff 0.75'':6
- Mate:758: Spacer (Nylon), 0.250'' (mod):2 ↔ Standoff 0.75'':7
- Mate:759: Spacer (Nylon), 0.250'':3 ↔ Standoff 0.75'':8
- Mate:760: Spacer (Nylon), 0.250'':3 ↔ Standoff 0.75'':8
- Mate:761: Spacer (Nylon), 0.250'' (mod):2 ↔ Standoff 0.75'':7
- Mate:762: Spacer (Thin), 4.6mm:4 ↔ Standoff 0.75'':6
- Mate:763: Spacer (Thin), 4.6mm:3 ↔ Standoff 0.75'':5
- Mate:764: Spacer (Nylon), 0.250'':1 ↔ Standoff 0.75'':3
- Mate:765: Spacer (Nylon), 0.250'' (mod):1 ↔ Standoff 0.75'':4
- Mate:766: Spacer (Thin), 4.6mm:1 ↔ Standoff 0.75'':1
- Mate:767: Spacer (Nylon), 0.250'':3 ↔ Screw 8-32 x 0.500''-Silver:7
- Mate:769: Standoff 0.75'':3 ↔ Screw 8-32 x 0.500''-Silver:9
- Mate:770: Spacer (Thin), 4.6mm:4 ↔ Screw 8-32 x 0.500''-Silver:10
- Mate:771: Spacer (Thin), 4.6mm:1 ↔ Screw 8-32 x 0.500''-Silver:14
- Mate:772: Spacer (Thin), 4.6mm:2 ↔ Screw 8-32 x 0.500''-Silver:12
- Mate:773: Spacer (Thin), 4.6mm:3 ↔ Screw 8-32 x 0.500''-Silver:11
- Mate:774: Standoff 0.75'':7 ↔ Screw 8-32 x 0.500''-Silver:13
- Mate:776: 5 x 2:1 ↔ Screw 8-32 x 0.500''-Silver:13
- Mate:777: 5 x 2:1 ↔ Screw 8-32 x 0.500''-Silver:7
- Mate:778: 5 x 2:1 ↔ Screw 8-32 x 0.500''-Silver:10
- Mate:779: 5 x 2:1 ↔ Screw 8-32 x 0.500''-Silver:11
- Mate:780: 5 x 2:1 ↔ Screw 8-32 x 0.500''-Silver:12
- Mate:781: Spacer (Thin), 4.6mm:2 ↔ Standoff 0.75'':2
- Mate:782: 5 x 2:1 ↔ Screw 8-32 x 0.500''-Silver:9
- Mate:783: 5 x 2:1 ↔ Screw 8-32 x 0.500''-Silver:8
- Mate:784: 1103 lift base:1 ↔ Standoff 0.75'':2
- Mate:785: 5 x 2:1 ↔ Screw 8-32 x 0.500''-Silver:14
- Tangent:219 (0.2311 mm): 1103 lift base:1 ↔ Standoff 0.75'':3
- Tangent:220 (0.2311 mm): 1103 lift base:1 ↔ Standoff 0.75'':3
- Mate:786: Standoff 0.75'':3 ↔ Screw 8-32 x 0.250''-Silver:9
- Mate:787: Standoff 0.75'':4 ↔ Screw 8-32 x 0.250''-Silver:10
- Mate:788: Standoff 0.75'':1 ↔ Screw 8-32 x 0.250''-Silver:11
- Mate:789: Standoff 0.75'':2 ↔ Screw 8-32 x 0.250''-Silver:12
- Mate:790: 1103 lift base:1 ↔ Screw 8-32 x 0.250''-Silver:9
- Mate:791: 1103 lift base:1 ↔ Screw 8-32 x 0.250''-Silver:10
- Mate:792: 1103 lift base:1 ↔ Screw 8-32 x 0.250''-Silver:12
- Mate:793: 1103 lift base:1 ↔ Screw 8-32 x 0.250''-Silver:11
- Mate:794: Standoff 0.75'':7 ↔ Screw 8-32 x 0.250''-Silver:13
- Mate:795: Standoff 0.75'':8 ↔ Screw 8-32 x 0.250''-Silver:14
- Mate:796: Standoff 0.75'':5 ↔ Screw 8-32 x 0.250''-Silver:15
- Mate:797: Standoff 0.75'':6 ↔ Screw 8-32 x 0.250''-Silver:16
- Mate:798: 1103 lift base:1 ↔ Screw 8-32 x 0.250''-Silver:15
- Mate:799: 1103 lift base:1 ↔ Screw 8-32 x 0.250''-Silver:13
- Mate:800: 1103 lift base:1 ↔ Screw 8-32 x 0.250''-Silver:14
- Mate:801: 1103 lift base:1 ↔ Screw 8-32 x 0.250''-Silver:16
- Mate:802: VEX-HINGE 4x RevA:1 ↔ VEX-HINGE-2 RevA_1:1
- Mate:803: VEX-HINGE 4x RevA:1 ↔ VEX-HINGE-2 RevA_1:1
- Tangent:222 (0.1905 mm): 1103 lift base:1 ↔ Bearing Flat (2-hole):1
- Tangent:223 (0.1905 mm): 1103 lift base:1 ↔ Bearing Flat (2-hole):1
- Tangent:224 (0.1905 mm): 1103 lift base:1 ↔ Bearing Flat (2-hole):1
- Mate:804: 1103 lift base:1 ↔ Bearing Flat (2-hole):1
- Mate:805: Bearing Flat (2-hole):1 ↔ Bearing Flat (2-hole):2
- Mate:806: 1103 lift base:1 ↔ Bearing Flat (2-hole):2
- Mate:807: Bearing Flat (2-hole):1 ↔ Bearing Flat (2-hole):2
- Mate:808: Bearing Flat (2-hole):1 ↔ .5'' Screw & Nylock Nut:1
- Mate:809: Bearing Flat (2-hole):2 ↔ .5'' Screw & Nylock Nut:2
- Mate:810: 1103 lift base:1 ↔ .5'' Screw & Nylock Nut:2
- Mate:811: Bearing Flat (2-hole):1 ↔ .5'' Screw & Nylock Nut:1
- Mate:812: Bearing Flat (2-hole):1 ↔ Spacer (Thin), 4.6mm:5
- Mate:813: Bearing Flat (2-hole):1 ↔ Spacer (Thin), 4.6mm:5
- Mate:814: Bearing Flat (2-hole):2 ↔ Spacer (Thin), 4.6mm:6
- Mate:815: Bearing Flat (2-hole):2 ↔ Spacer (Thin), 4.6mm:6
- Mate:816: 2 x 12:1 ↔ Bearing Assembly (end hole):2
- Mate:817 (2.3114 mm): 2 x 12:1 ↔ Bearing Assembly (end hole):2
- Mate:818 (2.3114 mm): 2 x 12:2 ↔ Bearing Assembly (both end holes):1
- Mate:819: 1103 sprocket3:1 ↔ 5 x 2:2
- Mate:820: 1103 lift base:1 ↔ Standoff 0.75'':3
- Mate:821: 5 x 2:1 ↔ Spacer (Nylon), 0.250'':1
- Mate:822: VEX-HINGE 4x RevA:1 ↔ 5 x 2:1
- Angle:1 (0 deg): 1103 lift base:1 ↔ 5 x 2:1
- Angle:2 (0 deg): 1103 lift base:1 ↔ VEX-HINGE 4x RevA:1
- [Mate]: Screw 8-32 x 0.375''-Silver:5 ↔ Spacer (Thin), 4.6mm:7
- [Mate]: Screw 8-32 x 0.375''-Silver:6 ↔ Spacer (Thin), 4.6mm:8
- [Mate]: Screw 8-32 x 0.375''-Silver:7 ↔ Spacer (Thin), 4.6mm:9
- [Mate]: Screw 8-32 x 0.375''-Silver:8 ↔ Spacer (Thin), 4.6mm:10
- Mate:827: 5 x 2:2 ↔ Spacer (Thin), 4.6mm:7
- Mate:828: 5 x 2:2 ↔ Spacer (Thin), 4.6mm:8
- Mate:829: 5 x 2:2 ↔ Spacer (Thin), 4.6mm:9
- Mate:830: 5 x 2:2 ↔ Spacer (Thin), 4.6mm:10
- Mate:831: 1103 sprocket2:1 ↔ Screw 8-32 x 0.375''-Silver:6
- Mate:832: Spacer (Thin), 4.6mm:6 ↔ Screw 8-32 x 0.875''-Silver:2
- Mate:833: Nut 8-32 Nylock:10 ↔ Screw 8-32 x 0.875''-Silver:2
- Mate:834 (1.6002 mm): Spacer (Thin), 4.6mm:6 ↔ Screw 8-32 x 0.875''-Silver:2
- Mate:835 (1.1684 mm): 1103 lift base:1 ↔ Nut 8-32 Nylock:10
- Mate:836: Spacer (Thin), 4.6mm:5 ↔ Screw 8-32 x 0.875''-Silver:3
- Mate:837 (1.6002 mm): Spacer (Thin), 4.6mm:5 ↔ Screw 8-32 x 0.875''-Silver:3
- Mate:838: Nut 8-32 Nylock:11 ↔ Screw 8-32 x 0.875''-Silver:3
- Mate:839 (1.1684 mm): 1103 lift base:1 ↔ Nut 8-32 Nylock:11
